# Autodesk Inventor assembly: Structure
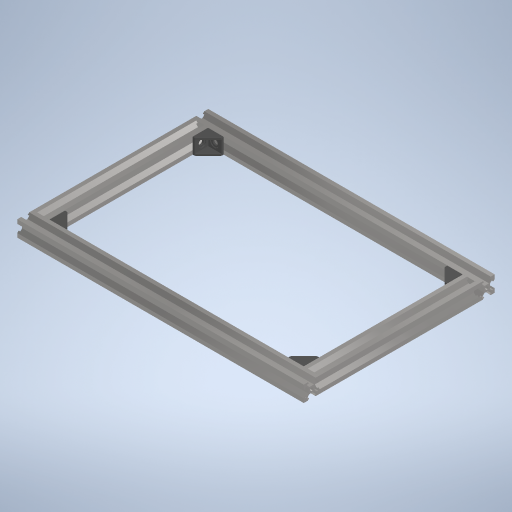
[picture p0: Inventor's stored thumbnail of the model, 512x512]
Saved by Autodesk Inventor 2024.2 (Build 282272000, 272)
## iProperties
Created: 2025-06-14
Part Number: Structure
Document SubType Name: Assembly
Designer: Admin
Author: Admin
## Documents named in this file (4)
- C:\Users\Admin\Documents\GitHub\ExplorateurErrant\Assemblies\Structure.iam
- C:\Users\Admin\Documents\GitHub\ExplorateurErrant\Estructura\ST-AluminumProfile-200.ipt
- C:\Users\Admin\Documents\GitHub\ExplorateurErrant\Estructura\ST-AluminumProfile-360.ipt
- C:\Users\Admin\Documents\GitHub\ExplorateurErrant\Estructura\ST-CornerBracket-2020.ipt
## Components (8 placed, 3 different names)
1. ST-AluminumProfile-200:1 — Mate:1, Flush:1, Flush:2, Mate:2, Mate:4, Flush:4, Flush:5, Mate:6
2. ST-AluminumProfile-360:1 — Mate:4, Flush:4, Flush:5, Mate:5, Flush:6, Mate:7, Flush:7, Flush:8, Mate:10, Flush:10
3. ST-AluminumProfile-360:2 — Mate:1, Flush:1, Flush:2, Mate:3, Flush:3, Mate:8, Flush:9
4. ST-CornerBracket-2020:1 — Mate:10, Mate:11, Flush:10
5. ST-CornerBracket-2020:2 — Mate:5, Mate:6, Flush:6
6. ST-CornerBracket-2020:3 — Mate:2, Mate:3, Flush:3
7. ST-CornerBracket-2020:4 — Mate:8, Mate:9, Flush:9
8. ST-AluminumProfile-200:2 — Mate:7, Flush:7, Flush:8, Mate:9, Mate:11
## Relationships (21: Mate 11, Flush 10)
- Mate:1: ST-AluminumProfile-200:1 ↔ ST-AluminumProfile-360:2
- Flush:1: ST-AluminumProfile-200:1 ↔ ST-AluminumProfile-360:2
- Flush:2: ST-AluminumProfile-200:1 ↔ ST-AluminumProfile-360:2
- Mate:2: ST-AluminumProfile-200:1 ↔ ST-CornerBracket-2020:3
- Mate:3: ST-AluminumProfile-360:2 ↔ ST-CornerBracket-2020:3
- Flush:3: ST-AluminumProfile-360:2 ↔ ST-CornerBracket-2020:3
- Mate:4: ST-AluminumProfile-200:1 ↔ ST-AluminumProfile-360:1
- Flush:4: ST-AluminumProfile-200:1 ↔ ST-AluminumProfile-360:1
- Flush:5: ST-AluminumProfile-200:1 ↔ ST-AluminumProfile-360:1
- Mate:5: ST-AluminumProfile-360:1 ↔ ST-CornerBracket-2020:2
- Mate:6: ST-AluminumProfile-200:1 ↔ ST-CornerBracket-2020:2
- Flush:6: ST-AluminumProfile-360:1 ↔ ST-CornerBracket-2020:2
- Mate:7: ST-AluminumProfile-360:1 ↔ ST-AluminumProfile-200:2
- Flush:7: ST-AluminumProfile-360:1 ↔ ST-AluminumProfile-200:2
- Flush:8: ST-AluminumProfile-360:1 ↔ ST-AluminumProfile-200:2
- Mate:8: ST-AluminumProfile-360:2 ↔ ST-CornerBracket-2020:4
- Mate:9: ST-CornerBracket-2020:4 ↔ ST-AluminumProfile-200:2
- Flush:9: ST-AluminumProfile-360:2 ↔ ST-CornerBracket-2020:4
- Mate:10: ST-AluminumProfile-360:1 ↔ ST-CornerBracket-2020:1
- Mate:11: ST-CornerBracket-2020:1 ↔ ST-AluminumProfile-200:2
- Flush:10: ST-AluminumProfile-360:1 ↔ ST-CornerBracket-2020:1
